# Autodesk Inventor assembly: robot arm box
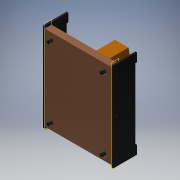
[picture p0: Inventor's stored thumbnail of the model, 180x180]
Saved by Autodesk Inventor 2018 (Build 220112000, 112)
## iProperties
Created: 2017-10-09
Part Number: robot arm box
Document SubType Name: Assembly
Designer: HP
Author: HP
## Documents named in this file (4)
- C:\!_Dani\!_cloud\ownCloud\rover\Robot arm box\robot arm box.iam
- C:\!_Dani\!_cloud\ownCloud\rover\Robot arm box\basic plate.ipt
- C:\!_Dani\!_cloud\ownCloud\rover\Robot arm box\sides.ipt
- C:\!_Dani\!_cloud\ownCloud\rover\Robot arm box\robot arm box parameters.xlsx
## Components (3 placed, 2 different names)
1. basic plate:1 — Flush:2, Mate:1, Mate:2, Flush:3, Flush:4, Mate:3, Flush:5
2. sides:1 — Flush:3, Flush:4, Flush:6
3. sides:2 — Mate:3, Flush:5, Flush:6
## Relationships (8: Flush 5, Mate 3)
- Flush:2: basic plate:1
- Mate:1: basic plate:1
- Mate:2: basic plate:1
- Flush:3: basic plate:1 ↔ sides:1
- Flush:4 (0.5 mm): basic plate:1 ↔ sides:1
- Mate:3 (0.5 mm): basic plate:1 ↔ sides:2
- Flush:5: basic plate:1 ↔ sides:2
- Flush:6: sides:1 ↔ sides:2
## Named parameters: plate_thickness = 5 mm, ABS_tolerance = 0.1 mm, laser_cutter_thickness = 0.1 mm, basic_plate_offset = 0.5 mm
